# Autodesk Inventor assembly: Plasma-vessel-with-plasma-box
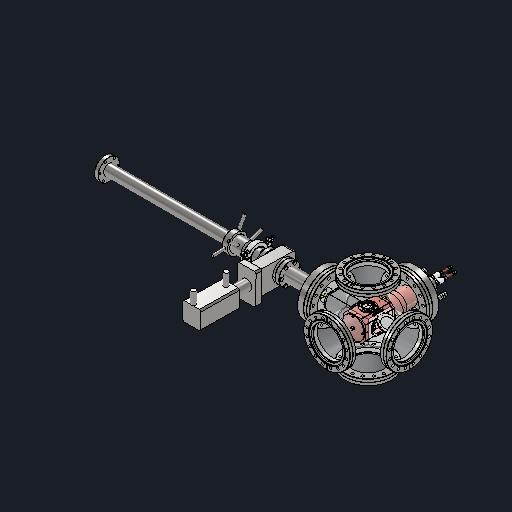
[picture p0: Inventor's stored thumbnail of the model, 512x512]
Saved by Autodesk Inventor 2027.1 (Build 311270010, 270A)
## iProperties
Created: 2024-05-09
Part Number: Plasma-vessel-with-plasma-box
Document SubType Name: Assembly
Designer: kuzmin
Mass: 19614.5 g
Surface Area: 13609.5 cm^2
Volume: 3689.47 cm^3
Density: 5.31636 g/cm^3
Author: kuzmin
## iProperties of the stored document MemberDocs/xM1vteul5Fszost223pdh0as2Dc
Created: 2024-05-09
Part Number: Plasma-vessel-with-plasma-box
Document SubType Name: Assembly
Designer: kuzmin
Mass: 19614.5 g
Surface Area: 13609.5 cm^2
Volume: 3689.47 cm^3
Density: 5.31636 g/cm^3
Author: kuzmin
## Documents named in this file (17)
- C:\Users\queezz\Dropbox\Drawings\pihti-cad\Plasma Vessel\Plasma-vessel-with-plasma-box.iam
- C:\Users\queezz\Dropbox\Drawings\pihti-cad\Plasma Vessel\Plasma-vacuum-cross\Plasma-vacuum-vessel-152IC-cross.iam
- C:\Users\queezz\Dropbox\Drawings\pihti-cad\Plasma Vessel\Plasma-Flange-2024\cathode-box-on-a-flange.iam
- C:\Users\queezz\Dropbox\Drawings\pihti-cad\Plasma Vessel\Cathode-Flange-Cage\CathodeCage.iam
- C:\Users\queezz\Dropbox\Drawings\pihti-cad\Plasma Vessel\Cathode-Anode-Flange\Cathode-Anode-70IC-flange-with-feeds.iam
- C:\Users\queezz\Dropbox\Drawings\pihti-cad\Plasma Vessel\Plasma-Box\Plasma-box-hayashi-aka-upgrade.iam
- C:\Users\queezz\Dropbox\Drawings\pihti-cad\ContentCenter\Fastners\M3x8-SHCS.ipt
- C:\Users\queezz\Dropbox\Drawings\pihti-cad\Plasma Vessel\Plasma-Box\probe-gate-with-spindel.iam
- C:\Users\queezz\Dropbox\Drawings\pihti-cad\Plasma Vessel\Cathode-Anode-Flange\cf70_spacer.ipt
- C:\Users\queezz\Dropbox\Drawings\pihti-cad\Plasma Vessel\Plasma-Box\anode-on-flange.iam
- C:\Users\queezz\Dropbox\Drawings\pihti-cad\Plasma Vessel\entrance-mesh-assembly.iam
- C:\Users\queezz\Dropbox\Drawings\pihti-cad\Plasma Vessel\Oring-probe-flange-with-GV.iam
- C:\Users\queezz\Dropbox\Drawings\pihti-cad\PALP\PALP-prototype.iam
- C:\Users\queezz\Dropbox\Drawings\pihti-cad\Plasma Vessel\probe-port-mesh-welded.iam
- C:\Users\queezz\Dropbox\Drawings\pihti-cad\Plasma Vessel\Mesh-mounting-help.ipt
- C:\Users\queezz\Dropbox\Drawings\pihti-cad\Plasma Vessel\Cathode-Flange-Cage\Short-Cage.iam
- C:\Users\queezz\Dropbox\Drawings\pihti-cad\BoronProbe\palp-boron-hybrid.iam
## Components (23 placed, 16 different names)
1. Plasma-vacuum-vessel-152IC-cross:1 [sub-assembly] — Mate:1, Flush:1, Flush:2, Rotational:1, Mate:15, Rigid:17
2. cathode-box-on-a-flange:1 [sub-assembly] — Rotational:1, Rotational:2, Mate:2, Mate:5, Rigid:10
3. CathodeCage:1 [sub-assembly] — Rotational:2
4. Cathode-Anode-70IC-flange-with-feeds:1 [sub-assembly] — Mate:2, Mate:5, Mate:6
5. Plasma-box-hayashi-aka-upgrade:1 [sub-assembly] — Mate:3, Mate:4, Hinge Angle, Mate:7, Mate:8, Mate:9, Mate:13, Mate:17
6. probe-gate-with-spindel:1 [sub-assembly] — Mate:3, Mate:4, Hinge Angle
7. cf70_spacer:1 — Rigid:10, Mate:6
8. anode-on-flange:1 [sub-assembly] — Mate:7, Mate:8, Mate:9, Rigid:11, Rigid:12, Rigid:13, Rigid:14
9. entrance-mesh-assembly:1 [sub-assembly] — Mate:13, Mate:17
10. Oring-probe-flange-with-GV:1 [sub-assembly] — Mate:15, Mate:18, Rigid:16, Mate:19
11. PALP-prototype:1 [sub-assembly] — Mate:18
12. probe-port-mesh-welded:1 [sub-assembly]
13. Mesh-mounting-help:1 — Rigid:16
14. Short-Cage:1 [sub-assembly] — Rigid:17
15. palp-boron-hybrid:1 [sub-assembly] — Mate:19
16. SS ISO 4762 M3 x 8:5 — Rigid:11
17. SS ISO 4762 M3 x 8:6 — Rigid:12
18. SS ISO 4762 M3 x 8:7 — Rigid:14
19. SS ISO 4762 M3 x 8:8 — Rigid:13
20. SS ISO 4762 M3 x 8:1
21. SS ISO 4762 M3 x 8:2
22. SS ISO 4762 M3 x 8:3
23. SS ISO 4762 M3 x 8:4
## Relationships (29: Mate 16, WeldJoint 8, Flush 2, RevoluteJoint 2, Angle 1)
- Mate:1: Plasma-vacuum-vessel-152IC-cross:1
- Flush:1: Plasma-vacuum-vessel-152IC-cross:1
- Flush:2: Plasma-vacuum-vessel-152IC-cross:1
- Rotational:1 [RevoluteJoint]: Plasma-vacuum-vessel-152IC-cross:1 ↔ cathode-box-on-a-flange:1
- Rotational:2 [RevoluteJoint]: cathode-box-on-a-flange:1 ↔ CathodeCage:1
- Mate:2: cathode-box-on-a-flange:1 ↔ Cathode-Anode-70IC-flange-with-feeds:1
- Mate:3: Plasma-box-hayashi-aka-upgrade:1 ↔ probe-gate-with-spindel:1
- Mate:4: Plasma-box-hayashi-aka-upgrade:1 ↔ probe-gate-with-spindel:1
- Hinge Angle [Angle] (45 deg): Plasma-box-hayashi-aka-upgrade:1 ↔ probe-gate-with-spindel:1
- Mate:5: cathode-box-on-a-flange:1 ↔ Cathode-Anode-70IC-flange-with-feeds:1
- Rigid:10 [WeldJoint]: cathode-box-on-a-flange:1 ↔ cf70_spacer:1
- Mate:6: Cathode-Anode-70IC-flange-with-feeds:1 ↔ cf70_spacer:1
- Mate:7: Plasma-box-hayashi-aka-upgrade:1 ↔ anode-on-flange:1
- Mate:8: Plasma-box-hayashi-aka-upgrade:1 ↔ anode-on-flange:1
- Mate:9: Plasma-box-hayashi-aka-upgrade:1 ↔ anode-on-flange:1
- Rigid:11 [WeldJoint]: anode-on-flange:1 ↔ SS ISO 4762 M3 x 8:5
- Rigid:12 [WeldJoint]: anode-on-flange:1 ↔ SS ISO 4762 M3 x 8:6
- Rigid:13 [WeldJoint]: anode-on-flange:1 ↔ SS ISO 4762 M3 x 8:8
- Rigid:14 [WeldJoint]: anode-on-flange:1 ↔ SS ISO 4762 M3 x 8:7
- [Mate]: Plasma-vacuum-vessel-152IC-cross:1 ↔ Oring-probe-flange-with-GV:1
- [Mate]: Plasma-vacuum-vessel-152IC-cross:1 ↔ Oring-probe-flange-with-GV:1
- Mate:13: Plasma-box-hayashi-aka-upgrade:1 ↔ entrance-mesh-assembly:1
- Mate:15: Plasma-vacuum-vessel-152IC-cross:1 ↔ Oring-probe-flange-with-GV:1
- Mate:17: Plasma-box-hayashi-aka-upgrade:1 ↔ entrance-mesh-assembly:1
- Mate:18: Oring-probe-flange-with-GV:1 ↔ PALP-prototype:1
- [WeldJoint]: Oring-probe-flange-with-GV:1 ↔ probe-port-mesh-welded:1
- Rigid:16 [WeldJoint]: Oring-probe-flange-with-GV:1 ↔ Mesh-mounting-help:1
- Rigid:17 [WeldJoint]: Plasma-vacuum-vessel-152IC-cross:1 ↔ Short-Cage:1
- Mate:19: Oring-probe-flange-with-GV:1 ↔ palp-boron-hybrid:1
